# Autodesk Inventor assembly: Tauchzelle
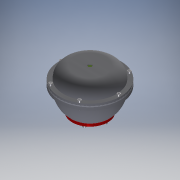
[picture p0: Inventor's stored thumbnail of the model, 180x180]
Saved by Autodesk Inventor 2016 (Build 200138000, 138)
## iProperties
Created: 2016-04-08
Part Number: Tauchzelle
Document SubType Name: Assembly
Designer: Johann
Author: Johann
## Documents named in this file (23)
- C:\Users\Johann\Documents\Uni\Bachelorarbeit\Inventor\Tauchzelle.iam
- C:\Users\Johann\Documents\Uni\Bachelorarbeit\Inventor\Oben_Schale.ipt
- C:\Users\Johann\Documents\Uni\Bachelorarbeit\Inventor\Unten_Schale.ipt
- C:\Users\Johann\Documents\Uni\Bachelorarbeit\Inventor\Drucksensor.ipt
- C:\Users\Johann\Documents\Uni\Bachelorarbeit\Inventor\BFA_30_25_10_530043_Rollmembran_mittel.ipt
- C:\Users\Johann\Documents\Uni\Bachelorarbeit\Inventor\GP17AAAH.ipt
- C:\Users\Johann\Documents\Uni\Bachelorarbeit\Inventor\Unten_Motor_Drehmomentuebertraeger.ipt
- C:\Users\Johann\Documents\Uni\Bachelorarbeit\Inventor\Motor_Faulhaber_mit_Getriebe.ipt
- C:\Users\Johann\Documents\Uni\Bachelorarbeit\Inventor\Unten_Welle.ipt
- C:\Users\Johann\Documents\Uni\Bachelorarbeit\Inventor\Unten_Zahnstange.ipt
- C:\Users\Johann\Documents\Uni\Bachelorarbeit\Inventor\Unten_Membran_Dichtring.ipt
- C:\Users\Johann\Documents\Uni\Bachelorarbeit\Inventor\Unten_Einsatz_opt.ipt
- C:\Users\Johann\Documents\Uni\Bachelorarbeit\Inventor\Halterung_Motor_gross.ipt
- C:\Users\Johann\Documents\Uni\Bachelorarbeit\Inventor\Halterung_Schalter.ipt
- C:\Users\Johann\Documents\Uni\Bachelorarbeit\Inventor\Platine.ipt
- C:\Users\Johann\Documents\Uni\Bachelorarbeit\Inventor\Unten_Abstandshalter.ipt
- C:\Users\Johann\Documents\Uni\Bachelorarbeit\Inventor\Dichtring.ipt
- C:\Users\Johann\Documents\Uni\Bachelorarbeit\Inventor\Teensy.ipt
- C:\Users\Johann\Documents\Uni\Bachelorarbeit\Inventor\DRV8834.ipt
- C:\Users\Johann\Documents\Inventor\Content Center Files\R2016\de-DE\ISO 4762(2)\ISO 4762 - M3 x 20ISO.ipt
- C:\Users\Johann\Documents\Inventor\Content Center Files\R2016\de-DE\ISO 4762(2)\ISO 4762 - M3 x 25ISO.ipt
- C:\Users\Johann\Documents\Inventor\Content Center Files\R2016\de-DE\ISO 4762(2)\ISO 4762 - M3 x 10ISO.ipt
- C:\Users\Johann\Documents\Inventor\Content Center Files\R2016\de-DE\ISO 4762(2)\ISO 4762 - M3 x 12ISO.ipt
## Components (45 placed, 22 different names)
1. Drucksensor:1 — Passend:22, Passend:23, Fluchtend:9
2. Oben_Schale:1 — Passend:1, Passend:2, Passend:3, Passend:22, Passend:23, Passend:84, Passend:86, Passend:88, Passend:90, Passend:92, Passend:94
3. Unten_Schale:1 — Fluchtend:1, Fluchtend:2, Fluchtend:3, Passend:1, Passend:2, Passend:3, Passend:4, Passend:5, Fluchtend:6, Fluchtend:7, Passend:24, Passend:25, Passend:26, Passend:60, Passend:61, Passend:62, Passend:71, Passend:73, Passend:75, Passend:77, Passend:79, Passend:81, Passend:83, Passend:85, Passend:87, Passend:89, Passend:91, Passend:93
4. Dichtring:1 — Passend:60, Passend:61, Passend:62
5. Unten_Einsatz_opt:1 — Passend:5, Fluchtend:6, Fluchtend:7, Passend:7, Passend:8, Passend:9, Passend:10, Passend:11, Passend:12, Passend:16, Passend:17, Passend:18, Passend:19, Passend:20, Passend:21, Passend:27, Passend:28, Passend:29, Passend:30, Passend:31, Passend:32, Passend:33, Passend:34, Passend:35, Passend:36, Passend:37, Passend:38, Passend:39, Passend:40, Passend:41, Passend:42, Passend:43, Passend:44, Passend:48, Passend:63, Passend:65, Passend:67, Passend:69
6. Unten_Abstandshalter:1 — Passend:50, Passend:51
7. Unten_Abstandshalter:2 — Passend:52, Passend:53
8. Unten_Abstandshalter:3 — Passend:56, Passend:57
9. Unten_Abstandshalter:4 — Passend:54, Passend:55
10. Platine:1 — Passend:48, Passend:49, Passend:58, Passend:59, Passend:64, Passend:66
11. Halterung_Schalter:1 — Passend:45, Passend:46, Passend:47, Passend:49, Passend:53, Passend:68, Passend:70
12. Teensy:1 — Passend:59
13. DRV8834:1 — Passend:58
14. ISO 4762 M3 x 12:1 — Passend:83, Passend:84
15. ISO 4762 M3 x 12:2 — Passend:85, Passend:86
16. ISO 4762 M3 x 12:3 — Passend:87, Passend:88
17. ISO 4762 M3 x 12:4 — Passend:89, Passend:90
18. ISO 4762 M3 x 12:5 — Passend:91, Passend:92
19. ISO 4762 M3 x 12:6 — Passend:93, Passend:94
20. ISO 4762 M3 x 20:1 — Passend:63, Passend:64
21. ISO 4762 M3 x 20:2 — Passend:65, Passend:66
22. ISO 4762 M3 x 25:1 — Passend:67, Passend:68
23. ISO 4762 M3 x 25:2 — Passend:69, Passend:70
24. ISO 4762 M3 x 10:1 — Passend:71, Passend:72
25. ISO 4762 M3 x 10:2 — Passend:73, Passend:74
26. ISO 4762 M3 x 10:3 — Passend:75, Passend:76
27. ISO 4762 M3 x 10:4 — Passend:77, Passend:78
28. ISO 4762 M3 x 10:5 — Passend:79, Passend:80
29. ISO 4762 M3 x 10:6 — Passend:81, Passend:82
30. Motor_Faulhaber_mit_Getriebe:1 — Winkel:10, Passend:13, Passend:14, Passend:16
31. Unten_Welle:1 — Fluchtend:8, Passend:9, Passend:15
32. Unten_Motor_Drehmomentuebertraeger:1 — Winkel:10, Passend:13, Passend:14, Passend:15
33. Halterung_Motor_gross:1 — Passend:17, Passend:18, Passend:19, Passend:27, Passend:28, Passend:46, Passend:50, Passend:51, Passend:52
34. Halterung_Motor_gross:2 — Passend:10, Passend:11, Passend:12, Passend:29, Passend:30, Passend:47, Passend:54, Passend:55, Passend:56, Passend:57
35. Unten_Zahnstange:1 — Passend:6, Passend:7, Passend:8, Fluchtend:8, Passend:45
36. BFA_30_25_10_530043_Rollmembran_mittel:1 — Passend:4, Fluchtend:4, Fluchtend:5, Passend:6
37. Unten_Membran_Dichtring:1 — Passend:24, Passend:25, Passend:26, Passend:72, Passend:74, Passend:76, Passend:78, Passend:80, Passend:82
38. GP17AAAH:1 — Passend:20, Passend:21
39. GP17AAAH:2 — Passend:31, Passend:32
40. GP17AAAH:3 — Passend:33, Passend:34
41. GP17AAAH:4 — Passend:35, Passend:36
42. GP17AAAH:5 — Passend:37, Passend:38
43. GP17AAAH:6 — Passend:39, Passend:40
44. GP17AAAH:7 — Passend:41, Passend:42
45. GP17AAAH:8 — Passend:43, Passend:44
## Relationships (104: Mate 94, Flush 9, Angle 1)
- Fluchtend:1 [Flush]: Unten_Schale:1
- Fluchtend:2 [Flush]: Unten_Schale:1
- Fluchtend:3 [Flush]: Unten_Schale:1
- Passend:1 [Mate]: Oben_Schale:1 ↔ Unten_Schale:1
- Passend:2 [Mate]: Oben_Schale:1 ↔ Unten_Schale:1
- Passend:3 [Mate]: Oben_Schale:1 ↔ Unten_Schale:1
- Passend:4 [Mate]: Unten_Schale:1 ↔ BFA_30_25_10_530043_Rollmembran_mittel:1
- Fluchtend:4 [Flush]: BFA_30_25_10_530043_Rollmembran_mittel:1
- Fluchtend:5 [Flush]: BFA_30_25_10_530043_Rollmembran_mittel:1
- Passend:5 [Mate]: Unten_Schale:1 ↔ Unten_Einsatz_opt:1
- Fluchtend:6 [Flush]: Unten_Schale:1 ↔ Unten_Einsatz_opt:1
- Fluchtend:7 [Flush]: Unten_Schale:1 ↔ Unten_Einsatz_opt:1
- Passend:6 [Mate]: Unten_Zahnstange:1 ↔ BFA_30_25_10_530043_Rollmembran_mittel:1
- Passend:7 [Mate]: Unten_Einsatz_opt:1 ↔ Unten_Zahnstange:1
- Passend:8 [Mate]: Unten_Einsatz_opt:1 ↔ Unten_Zahnstange:1
- Fluchtend:8 [Flush]: Unten_Welle:1 ↔ Unten_Zahnstange:1
- Passend:9 [Mate]: Unten_Einsatz_opt:1 ↔ Unten_Welle:1
- Passend:10 [Mate]: Unten_Einsatz_opt:1 ↔ Halterung_Motor_gross:2
- Passend:11 [Mate]: Unten_Einsatz_opt:1 ↔ Halterung_Motor_gross:2
- Passend:12 [Mate]: Unten_Einsatz_opt:1 ↔ Halterung_Motor_gross:2
- Winkel:10 [Angle] (0 deg): Motor_Faulhaber_mit_Getriebe:1 ↔ Unten_Motor_Drehmomentuebertraeger:1
- Passend:13 [Mate]: Motor_Faulhaber_mit_Getriebe:1 ↔ Unten_Motor_Drehmomentuebertraeger:1
- Passend:14 [Mate]: Motor_Faulhaber_mit_Getriebe:1 ↔ Unten_Motor_Drehmomentuebertraeger:1
- Passend:15 [Mate]: Unten_Welle:1 ↔ Unten_Motor_Drehmomentuebertraeger:1
- Passend:16 [Mate]: Unten_Einsatz_opt:1 ↔ Motor_Faulhaber_mit_Getriebe:1
- Passend:17 [Mate]: Unten_Einsatz_opt:1 ↔ Halterung_Motor_gross:1
- Passend:18 [Mate]: Unten_Einsatz_opt:1 ↔ Halterung_Motor_gross:1
- Passend:19 [Mate]: Unten_Einsatz_opt:1 ↔ Halterung_Motor_gross:1
- Passend:20 [Mate]: Unten_Einsatz_opt:1 ↔ GP17AAAH:1
- Passend:21 [Mate]: Unten_Einsatz_opt:1 ↔ GP17AAAH:1
- Passend:22 [Mate]: Drucksensor:1 ↔ Oben_Schale:1
- Passend:23 [Mate]: Drucksensor:1 ↔ Oben_Schale:1
- Fluchtend:9 [Flush]: Drucksensor:1
- Passend:24 [Mate]: Unten_Schale:1 ↔ Unten_Membran_Dichtring:1
- Passend:25 [Mate]: Unten_Schale:1 ↔ Unten_Membran_Dichtring:1
- Passend:26 [Mate]: Unten_Schale:1 ↔ Unten_Membran_Dichtring:1
- Passend:27 [Mate]: Unten_Einsatz_opt:1 ↔ Halterung_Motor_gross:1
- Passend:28 [Mate]: Unten_Einsatz_opt:1 ↔ Halterung_Motor_gross:1
- Passend:29 [Mate]: Unten_Einsatz_opt:1 ↔ Halterung_Motor_gross:2
- Passend:30 [Mate]: Unten_Einsatz_opt:1 ↔ Halterung_Motor_gross:2
- Passend:31 [Mate]: Unten_Einsatz_opt:1 ↔ GP17AAAH:2
- Passend:32 [Mate]: Unten_Einsatz_opt:1 ↔ GP17AAAH:2
- Passend:33 [Mate]: Unten_Einsatz_opt:1 ↔ GP17AAAH:3
- Passend:34 [Mate]: Unten_Einsatz_opt:1 ↔ GP17AAAH:3
- Passend:35 [Mate]: Unten_Einsatz_opt:1 ↔ GP17AAAH:4
- Passend:36 [Mate]: Unten_Einsatz_opt:1 ↔ GP17AAAH:4
- Passend:37 [Mate]: Unten_Einsatz_opt:1 ↔ GP17AAAH:5
- Passend:38 [Mate]: Unten_Einsatz_opt:1 ↔ GP17AAAH:5
- Passend:39 [Mate]: Unten_Einsatz_opt:1 ↔ GP17AAAH:6
- Passend:40 [Mate]: Unten_Einsatz_opt:1 ↔ GP17AAAH:6
- Passend:41 [Mate]: Unten_Einsatz_opt:1 ↔ GP17AAAH:7
- Passend:42 [Mate]: Unten_Einsatz_opt:1 ↔ GP17AAAH:7
- Passend:43 [Mate]: Unten_Einsatz_opt:1 ↔ GP17AAAH:8
- Passend:44 [Mate]: Unten_Einsatz_opt:1 ↔ GP17AAAH:8
- Passend:45 [Mate] (9 mm): Halterung_Schalter:1 ↔ Unten_Zahnstange:1
- Passend:46 [Mate]: Halterung_Schalter:1 ↔ Halterung_Motor_gross:1
- Passend:47 [Mate]: Halterung_Schalter:1 ↔ Halterung_Motor_gross:2
- Passend:48 [Mate]: Unten_Einsatz_opt:1 ↔ Platine:1
- Passend:49 [Mate]: Platine:1 ↔ Halterung_Schalter:1
- Passend:50 [Mate]: Unten_Abstandshalter:1 ↔ Halterung_Motor_gross:1
- Passend:51 [Mate]: Unten_Abstandshalter:1 ↔ Halterung_Motor_gross:1
- Passend:52 [Mate]: Unten_Abstandshalter:2 ↔ Halterung_Motor_gross:1
- Passend:53 [Mate]: Unten_Abstandshalter:2 ↔ Halterung_Schalter:1
- Passend:54 [Mate]: Unten_Abstandshalter:4 ↔ Halterung_Motor_gross:2
- Passend:55 [Mate]: Unten_Abstandshalter:4 ↔ Halterung_Motor_gross:2
- Passend:56 [Mate]: Unten_Abstandshalter:3 ↔ Halterung_Motor_gross:2
- Passend:57 [Mate]: Unten_Abstandshalter:3 ↔ Halterung_Motor_gross:2
- Passend:58 [Mate]: Platine:1 ↔ DRV8834:1
- Passend:59 [Mate] (5 mm): Platine:1 ↔ Teensy:1
- Passend:60 [Mate]: Unten_Schale:1 ↔ Dichtring:1
- Passend:61 [Mate]: Unten_Schale:1 ↔ Dichtring:1
- Passend:62 [Mate]: Unten_Schale:1 ↔ Dichtring:1
- Passend:63 [Mate]: Unten_Einsatz_opt:1 ↔ ISO 4762 M3 x 20:1
- Passend:64 [Mate]: Platine:1 ↔ ISO 4762 M3 x 20:1
- Passend:65 [Mate]: Unten_Einsatz_opt:1 ↔ ISO 4762 M3 x 20:2
- Passend:66 [Mate]: Platine:1 ↔ ISO 4762 M3 x 20:2
- Passend:67 [Mate]: Unten_Einsatz_opt:1 ↔ ISO 4762 M3 x 25:1
- Passend:68 [Mate]: Halterung_Schalter:1 ↔ ISO 4762 M3 x 25:1
- Passend:69 [Mate]: Unten_Einsatz_opt:1 ↔ ISO 4762 M3 x 25:2
- Passend:70 [Mate]: Halterung_Schalter:1 ↔ ISO 4762 M3 x 25:2
- Passend:71 [Mate]: Unten_Schale:1 ↔ ISO 4762 M3 x 10:1
- Passend:72 [Mate]: ISO 4762 M3 x 10:1 ↔ Unten_Membran_Dichtring:1
- Passend:73 [Mate]: Unten_Schale:1 ↔ ISO 4762 M3 x 10:2
- Passend:74 [Mate]: ISO 4762 M3 x 10:2 ↔ Unten_Membran_Dichtring:1
- Passend:75 [Mate]: Unten_Schale:1 ↔ ISO 4762 M3 x 10:3
- Passend:76 [Mate]: ISO 4762 M3 x 10:3 ↔ Unten_Membran_Dichtring:1
- Passend:77 [Mate]: Unten_Schale:1 ↔ ISO 4762 M3 x 10:4
- Passend:78 [Mate]: ISO 4762 M3 x 10:4 ↔ Unten_Membran_Dichtring:1
- Passend:79 [Mate]: Unten_Schale:1 ↔ ISO 4762 M3 x 10:5
- Passend:80 [Mate]: ISO 4762 M3 x 10:5 ↔ Unten_Membran_Dichtring:1
- Passend:81 [Mate]: Unten_Schale:1 ↔ ISO 4762 M3 x 10:6
- Passend:82 [Mate]: ISO 4762 M3 x 10:6 ↔ Unten_Membran_Dichtring:1
- Passend:83 [Mate]: Unten_Schale:1 ↔ ISO 4762 M3 x 12:1
- Passend:84 [Mate]: Oben_Schale:1 ↔ ISO 4762 M3 x 12:1
- Passend:85 [Mate]: Unten_Schale:1 ↔ ISO 4762 M3 x 12:2
- Passend:86 [Mate]: Oben_Schale:1 ↔ ISO 4762 M3 x 12:2
- Passend:87 [Mate]: Unten_Schale:1 ↔ ISO 4762 M3 x 12:3
- Passend:88 [Mate]: Oben_Schale:1 ↔ ISO 4762 M3 x 12:3
- Passend:89 [Mate]: Unten_Schale:1 ↔ ISO 4762 M3 x 12:4
- Passend:90 [Mate]: Oben_Schale:1 ↔ ISO 4762 M3 x 12:4
- Passend:91 [Mate]: Unten_Schale:1 ↔ ISO 4762 M3 x 12:5
- Passend:92 [Mate]: Oben_Schale:1 ↔ ISO 4762 M3 x 12:5
- Passend:93 [Mate]: Unten_Schale:1 ↔ ISO 4762 M3 x 12:6
- Passend:94 [Mate]: Oben_Schale:1 ↔ ISO 4762 M3 x 12:6
